# Autodesk Inventor assembly: Glovebox_with_rings
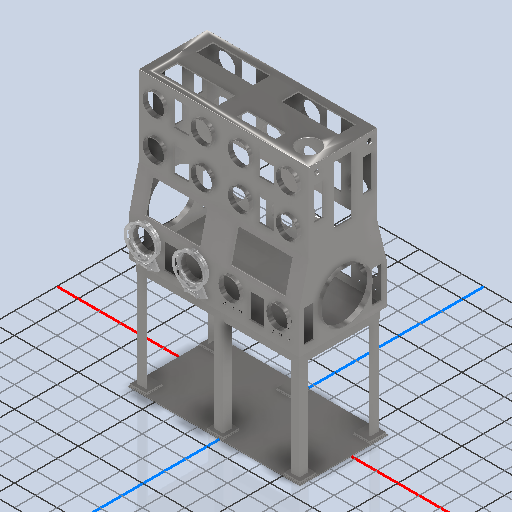
[picture p0: Inventor's stored thumbnail of the model, 512x512]
Saved by Autodesk Inventor 2026.1 (Build 301233000, 233)
## iProperties
Created: 2025-08-31
Part Number: Glovebox_with_rings
Document SubType Name: Assembly
Designer: baseb
Author: baseb
## Documents named in this file (3)
- C:\Users\baseb\Desktop\LANL-Glovebox-Closure-Mechanism\Glovebox_with_rings.iam
- C:\Users\baseb\Desktop\LANL-Glovebox-Closure-Mechanism\Glovebox 3D Model Updated.ipt
- C:\Users\baseb\Desktop\LANL-Glovebox-Closure-Mechanism\ring_assembly.iam
## Components (3 placed, 2 different names)
1. Glovebox 3D Model Updated:1 — Mate:1, Mate:2, Mate:3, Mate:4
2. ring_assembly:1 [sub-assembly] — Mate:1, Mate:2
3. ring_assembly:2 [sub-assembly] — Mate:3, Mate:4
## Relationships (4: Mate 4)
- Mate:1: Glovebox 3D Model Updated:1 ↔ ring_assembly:1
- Mate:2: Glovebox 3D Model Updated:1 ↔ ring_assembly:1
- Mate:3: Glovebox 3D Model Updated:1 ↔ ring_assembly:2
- Mate:4: Glovebox 3D Model Updated:1 ↔ ring_assembly:2
